# Autodesk Inventor assembly: leg_assembly
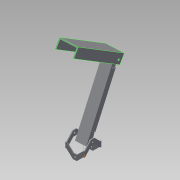
[picture p0: Inventor's stored thumbnail of the model, 180x180]
Saved by Autodesk Inventor 2015 (Build 190159000, 159)
## iProperties
Created: 2014-06-09
Part Number: leg_assembly
Document SubType Name: Assembly
Designer: L
Author: L
## Documents named in this file (4)
- D:\Documents\Autocad\leg_assembly.iam
- D:\Documents\Autocad\shoulder_servo_joint.ipt
- D:\Documents\Autocad\upper_leg.iam
- D:\Documents\Autocad\lower_leg.ipt
## Components (3 placed, 3 different names)
1. shoulder_servo_joint:1 — Mate:1, Mate:2, Mate:5
2. upper_leg:1 [sub-assembly] — Mate:1, Mate:2, Mate:3, Mate:4
3. lower_leg:1 — Mate:3, Mate:4
## Relationships (5: Mate 5)
- Mate:1: shoulder_servo_joint:1 ↔ upper_leg:1
- Mate:2: shoulder_servo_joint:1 ↔ upper_leg:1
- Mate:3: upper_leg:1 ↔ lower_leg:1
- Mate:4: upper_leg:1 ↔ lower_leg:1
- Mate:5: shoulder_servo_joint:1
